# Autodesk Inventor assembly: piercable_septum
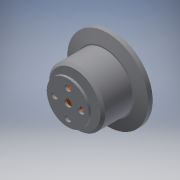
[picture p0: Inventor's stored thumbnail of the model, 180x180]
Saved by Autodesk Inventor 2019.4 (Build 234330000, 330)
## iProperties
Created: 2021-04-23
Part Number: piercable_septum
Document SubType Name: Assembly
Designer: PattersonOfficeMini
Author: PattersonOfficeMini
## Documents named in this file (4)
- C:\Users\PattersonOfficeMini\Dropbox\Lincolndocs\piercable_septum.iam
- C:\Users\PattersonOfficeMini\Dropbox\Lincolndocs\piercable_septum_flange.ipt
- C:\Users\PattersonOfficeMini\Dropbox\Lincolndocs\piercable_septum_clamp.ipt
- C:\Users\PattersonOfficeMini\Dropbox\Lincolndocs\septum.ipt
## Components (3 placed, 3 different names)
1. piercable_septum_flange:1 — Mate:1, Mate:2, Mate:3
2. piercable_septum_clamp:1 — Mate:1, Mate:2
3. septum:1 — Mate:3
## Relationships (3: Mate 3)
- Mate:1: piercable_septum_flange:1 ↔ piercable_septum_clamp:1
- Mate:2: piercable_septum_flange:1 ↔ piercable_septum_clamp:1
- Mate:3: piercable_septum_flange:1 ↔ septum:1
